# Autodesk Inventor assembly: sus1
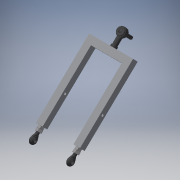
[picture p0: Inventor's stored thumbnail of the model, 180x180]
Saved by Autodesk Inventor 2018 (Build 220112000, 112)
## iProperties
Created: 2017-09-08
Part Number: sus1
Material: 一般
Document SubType Name: Assembly
Designer: mura5
Author: mura5
## Documents named in this file (6)
- C:\Users\Kenta\Documents\workspace\rbbr\cart\A.iam
- C:\Users\Kenta\Documents\workspace\rbbr\cart\Rod1.iam
- C:\Users\Kenta\Documents\workspace\rbbr\cart\iko_POS_14EC\AIS2016\POS 14ECBall.ipt
- C:\Users\Kenta\Documents\workspace\rbbr\cart\iko_LHSA_14\AIS2016\LHSA 14 Body1.ipt
- C:\Users\Kenta\Documents\workspace\rbbr\cart\iko_LHSA_14\AIS2016\LHSA 14 Body2.ipt
- C:\Users\Kenta\Documents\workspace\rbbr\cart\Pipe2.ipt
## Components (7 placed, 5 different names)
1. POS 14ECBall:1 — 回転:1, メイト:9, ボール:4
2. Rod1:1 [sub-assembly] — ボール:4, メイト:10, リジッド:4, 角度:1
3. Rod1:2 [sub-assembly] — ボール:2, リジッド:5
4. POS 14ECBall:2 — ボール:2, 回転:1, メイト:9
5. LHSA 14 Body1:1 — ボール:3, リジッド:3
6. LHSA 14 Body2:1 — ボール:3
7. Pipe2:1 — リジッド:3, メイト:10, リジッド:4, リジッド:5, 角度:2
## Relationships (11: BallJoint 3, WeldJoint 3, Mate 2, Angle 2, RevoluteJoint 1)
- ボール:2 [BallJoint]: Rod1:2 ↔ POS 14ECBall:2
- 回転:1 [RevoluteJoint] (200 mm): POS 14ECBall:1 ↔ POS 14ECBall:2
- ボール:3 [BallJoint]: LHSA 14 Body1:1 ↔ LHSA 14 Body2:1
- メイト:9 [Mate] (200 mm): POS 14ECBall:1 ↔ POS 14ECBall:2
- ボール:4 [BallJoint]: POS 14ECBall:1 ↔ Rod1:1
- リジッド:3 [WeldJoint]: LHSA 14 Body1:1 ↔ Pipe2:1
- メイト:10 [Mate]: Rod1:1 ↔ Pipe2:1
- リジッド:4 [WeldJoint]: Rod1:1 ↔ Pipe2:1
- リジッド:5 [WeldJoint]: Rod1:2 ↔ Pipe2:1
- 角度:1 [Angle] (0 deg): Rod1:1
- 角度:2 [Angle] (0 deg): Pipe2:1
